# Autodesk Inventor assembly: Assembly1
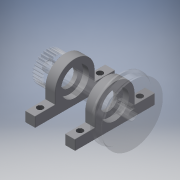
[picture p0: Inventor's stored thumbnail of the model, 180x180]
Saved by Autodesk Inventor 2019.1 (Build 231200000, 200)
## iProperties
Created: 2024-03-28
Part Number: Assembly1
Document SubType Name: Assembly
Designer: clariheelen
Author: clariheelen
## Documents named in this file (6)
- D:\Users\clari\Desktop\lucia\Landivar\Ciclo 7 (semestre 1)\Dinámica\Laboratorio\Intro Ensamble\Assembly1.iam
- D:\Users\clari\Desktop\lucia\Landivar\Ciclo 7 (semestre 1)\Dinámica\Laboratorio\Intro Ensamble\CUÑA.ipt
- D:\Users\clari\Desktop\lucia\Landivar\Ciclo 7 (semestre 1)\Dinámica\Laboratorio\Intro Ensamble\EJE_CUÑEROS (1).ipt
- D:\Users\clari\Desktop\lucia\Landivar\Ciclo 7 (semestre 1)\Dinámica\Laboratorio\Intro Ensamble\Ensamble.ipt
- D:\Users\clari\Desktop\lucia\Landivar\Ciclo 7 (semestre 1)\Dinámica\Laboratorio\Intro Ensamble\POLEA.ipt
- D:\Users\clari\Desktop\lucia\Landivar\Ciclo 7 (semestre 1)\Dinámica\Laboratorio\Intro Ensamble\Chumacera (pieza extra).ipt
## Components (6 placed, 5 different names)
1. EJE_CUÑEROS (1):1 — Mate:4, Mate:6, Mate:10, Flush:1, Cylindrical:1, Flush:2, Mate:13, Tangent:1, Mate:14, Tangent:2
2. POLEA:1 — Mate:1, Mate:2, Mate:3, Mate:11, Flush:1, Mate:12
3. CUÑA:1 — Mate:1, Mate:2, Mate:3, Mate:4, Mate:6, Mate:10, Mate:11, Mate:12
4. Ensamble:1 — Cylindrical:1, Flush:2
5. Chumacera (pieza extra):1 — Mate:13, Tangent:1, Flush:3
6. Chumacera (pieza extra):2 — Mate:14, Tangent:2, Flush:3
## Relationships (16: Mate 10, Flush 3, Tangent 2, CylindricalJoint 1)
- Mate:1: POLEA:1 ↔ CUÑA:1
- Mate:2: POLEA:1 ↔ CUÑA:1
- Mate:3: POLEA:1 ↔ CUÑA:1
- Mate:4: EJE_CUÑEROS (1):1 ↔ CUÑA:1
- Mate:6: EJE_CUÑEROS (1):1 ↔ CUÑA:1
- Mate:10: EJE_CUÑEROS (1):1 ↔ CUÑA:1
- Mate:11: POLEA:1 ↔ CUÑA:1
- Flush:1: EJE_CUÑEROS (1):1 ↔ POLEA:1
- Mate:12: POLEA:1 ↔ CUÑA:1
- Cylindrical:1: EJE_CUÑEROS (1):1 ↔ Ensamble:1
- Flush:2: EJE_CUÑEROS (1):1 ↔ Ensamble:1
- Mate:13: EJE_CUÑEROS (1):1 ↔ Chumacera (pieza extra):1
- Tangent:1: EJE_CUÑEROS (1):1 ↔ Chumacera (pieza extra):1
- Mate:14: EJE_CUÑEROS (1):1 ↔ Chumacera (pieza extra):2
- Tangent:2: EJE_CUÑEROS (1):1 ↔ Chumacera (pieza extra):2
- Flush:3: Chumacera (pieza extra):1 ↔ Chumacera (pieza extra):2
